# Autodesk Inventor assembly: Timing_Assy 4 Lanes
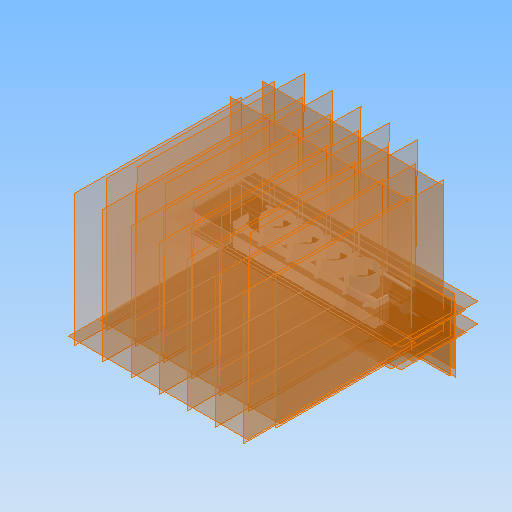
[picture p0: Inventor's stored thumbnail of the model, 512x512]
Saved by Autodesk Inventor 2018.1 (Build 221171000, 171)
## iProperties
Created: 2019-02-11
Part Number: Timing_Assy 4 Lanes
Document SubType Name: Assembly
Designer: James
Author: James
## Documents named in this file (9)
- C:\Users\admin\Desktop\Ball-Machine\Timing Gate\Timing - 4 Lanes\Timing_Assy 4 Lanes.iam
- C:\Users\admin\Desktop\Ball-Machine\Timing Gate\Nyloc Nut - M4.ipt
- C:\Users\admin\Desktop\Ball-Machine\Timing Gate\Socket Csk Screw - (A2) - M4 x  16.ipt
- C:\Users\admin\Desktop\Ball-Machine\Timing Gate\Timing_Angle Bracket.ipt
- C:\Users\admin\Desktop\Ball-Machine\Timing Gate\Socket Cap Screw - Standard - (A2) - M4 x 16.ipt
- C:\Users\admin\Desktop\Ball-Machine\Timing Gate\Timing_PVC Pipe.ipt
- C:\Users\admin\Desktop\Ball-Machine\Timing Gate\Timing - 4 Lanes\Timing_Backboard 4 Lanes.ipt
- C:\Users\admin\Desktop\Ball-Machine\Timing Gate\Timing - 4 Lanes\Timing_Assy_Lever Shaft 4 Lanes.iam
- C:\Users\admin\Desktop\Ball-Machine\Timing Gate\Timing - 4 Lanes\Timing_Assy_Star Shaft 4 Lanes.iam
## Components (33 placed, 8 different names)
1. Timing_Backboard 4 Lanes:1 — Flush:18, Mate:51, Mate:52, Tangent:1, Flush:19, Flush:20, Mate:55, Mate:56, Mate:59, Mate:60, Mate:67, Mate:68, Mate:69, Flush:27, Flush:28, Mate:74, Mate:75, Flush:29, Mate:82, Flush:30, Mate:83, Mate:84, Mate:85, Flush:31, Angle:2
2. Timing_Angle Bracket:1 — Mate:67, Mate:68, Mate:69, Flush:27, Flush:28, Mate:70, Mate:71, Mate:72, Mate:73, Flush:32, Flush:34
3. Nyloc Nut - M4:13 — Mate:74, Mate:76
4. Socket Cap Screw - Standard - (A2) - M4 x 16:3 — Mate:72, Mate:73, Mate:77
5. Nyloc Nut - M4:14 — Mate:75, Mate:77
6. Socket Cap Screw - Standard - (A2) - M4 x 16:4 — Mate:70, Mate:71, Mate:76
7. Timing_Angle Bracket:2 — Flush:29, Mate:82, Flush:30, Mate:83, Flush:33
8. Socket Cap Screw - Standard - (A2) - M4 x 16:5 — Mate:87
9. Socket Cap Screw - Standard - (A2) - M4 x 16:6 — Mate:86
10. Nyloc Nut - M4:15 — Mate:84, Mate:87
11. Nyloc Nut - M4:16 — Mate:85, Mate:86
12. Timing_Assy_Lever Shaft 4 Lanes:1 [sub-assembly] — Mate:88, Mate:89, Flush:31, Flush:32
13. Timing_Assy_Star Shaft 4 Lanes:1 [sub-assembly] — Flush:33, Flush:34, Mate:91, Angle:2, Mate:92
14. Timing_PVC Pipe:1 — Angle:1, Mate:51, Mate:52, Tangent:1, Mate:54
15. Nyloc Nut - M4:1 — Mate:58, Mate:59
16. Socket Csk Screw - (A2) - M4 x  16:1 — Mate:54, Mate:55, Flush:21, Mate:57
17. Socket Csk Screw - (A2) - M4 x  16:2 — Flush:21, Mate:56, Mate:58
18. Nyloc Nut - M4:2 — Mate:57, Mate:60
19. Timing_PVC Pipe:2
20. Nyloc Nut - M4:3
21. Socket Csk Screw - (A2) - M4 x  16:3
22. Socket Csk Screw - (A2) - M4 x  16:7
23. Nyloc Nut - M4:7
24. Timing_PVC Pipe:3
25. Nyloc Nut - M4:4
26. Socket Csk Screw - (A2) - M4 x  16:4
27. Socket Csk Screw - (A2) - M4 x  16:8
28. Nyloc Nut - M4:8
29. Timing_PVC Pipe:4
30. Nyloc Nut - M4:5
31. Socket Csk Screw - (A2) - M4 x  16:5
32. Socket Csk Screw - (A2) - M4 x  16:9
33. Nyloc Nut - M4:9
## Component patterns: (4 elements, first: Timing_PVC Pipe:1 + Nyloc Nut - M4:1 + Socket Csk Screw - (A2) - M4 x  16:1 + Socket Csk Screw - (A2) - M4 x  16:2 + Nyloc Nut - M4:2)
## Relationships (52: Mate 34, Flush 15, Angle 2, Tangent 1)
- Angle:1 (180 deg): Timing_PVC Pipe:1
- Flush:11 (-57.5 mm)
- Flush:12 (-5 mm)
- Flush:13 (30 mm)
- Flush:18: Timing_Backboard 4 Lanes:1
- Mate:51: Timing_Backboard 4 Lanes:1 ↔ Timing_PVC Pipe:1
- Mate:52: Timing_Backboard 4 Lanes:1 ↔ Timing_PVC Pipe:1
- Tangent:1: Timing_Backboard 4 Lanes:1 ↔ Timing_PVC Pipe:1
- Flush:19: Timing_Backboard 4 Lanes:1
- Flush:20: Timing_Backboard 4 Lanes:1
- Mate:54: Timing_PVC Pipe:1 ↔ Socket Csk Screw - (A2) - M4 x  16:1
- Mate:55 (-10.3 mm): Timing_Backboard 4 Lanes:1 ↔ Socket Csk Screw - (A2) - M4 x  16:1
- Flush:21: Socket Csk Screw - (A2) - M4 x  16:1 ↔ Socket Csk Screw - (A2) - M4 x  16:2
- Mate:56: Timing_Backboard 4 Lanes:1 ↔ Socket Csk Screw - (A2) - M4 x  16:2
- Mate:57: Socket Csk Screw - (A2) - M4 x  16:1 ↔ Nyloc Nut - M4:2
- Mate:58: Nyloc Nut - M4:1 ↔ Socket Csk Screw - (A2) - M4 x  16:2
- Mate:59: Timing_Backboard 4 Lanes:1 ↔ Nyloc Nut - M4:1
- Mate:60: Timing_Backboard 4 Lanes:1 ↔ Nyloc Nut - M4:2
- Mate:67: Timing_Backboard 4 Lanes:1 ↔ Timing_Angle Bracket:1
- Mate:68: Timing_Backboard 4 Lanes:1 ↔ Timing_Angle Bracket:1
- Mate:69: Timing_Backboard 4 Lanes:1 ↔ Timing_Angle Bracket:1
- Flush:27: Timing_Backboard 4 Lanes:1 ↔ Timing_Angle Bracket:1
- Flush:28: Timing_Backboard 4 Lanes:1 ↔ Timing_Angle Bracket:1
- Mate:70: Timing_Angle Bracket:1 ↔ Socket Cap Screw - Standard - (A2) - M4 x 16:4
- Mate:71: Timing_Angle Bracket:1 ↔ Socket Cap Screw - Standard - (A2) - M4 x 16:4
- Mate:72: Timing_Angle Bracket:1 ↔ Socket Cap Screw - Standard - (A2) - M4 x 16:3
- Mate:73: Timing_Angle Bracket:1 ↔ Socket Cap Screw - Standard - (A2) - M4 x 16:3
- Mate:74: Timing_Backboard 4 Lanes:1 ↔ Nyloc Nut - M4:13
- Mate:75: Timing_Backboard 4 Lanes:1 ↔ Nyloc Nut - M4:14
- Mate:76: Nyloc Nut - M4:13 ↔ Socket Cap Screw - Standard - (A2) - M4 x 16:4
- Mate:77: Socket Cap Screw - Standard - (A2) - M4 x 16:3 ↔ Nyloc Nut - M4:14
- [Mate]: Timing_Angle Bracket:2 ↔ Socket Cap Screw - Standard - (A2) - M4 x 16:6
- [Mate]: Timing_Angle Bracket:2 ↔ Socket Cap Screw - Standard - (A2) - M4 x 16:6
- [Mate]: Timing_Angle Bracket:2 ↔ Socket Cap Screw - Standard - (A2) - M4 x 16:5
- [Mate]: Timing_Angle Bracket:2 ↔ Socket Cap Screw - Standard - (A2) - M4 x 16:5
- Flush:29: Timing_Backboard 4 Lanes:1 ↔ Timing_Angle Bracket:2
- Mate:82: Timing_Backboard 4 Lanes:1 ↔ Timing_Angle Bracket:2
- Flush:30: Timing_Backboard 4 Lanes:1 ↔ Timing_Angle Bracket:2
- Mate:83: Timing_Backboard 4 Lanes:1 ↔ Timing_Angle Bracket:2
- Mate:84: Timing_Backboard 4 Lanes:1 ↔ Nyloc Nut - M4:15
- Mate:85: Timing_Backboard 4 Lanes:1 ↔ Nyloc Nut - M4:16
- Mate:86: Socket Cap Screw - Standard - (A2) - M4 x 16:6 ↔ Nyloc Nut - M4:16
- Mate:87: Socket Cap Screw - Standard - (A2) - M4 x 16:5 ↔ Nyloc Nut - M4:15
- Mate:88: Timing_Assy_Lever Shaft 4 Lanes:1
- Mate:89: Timing_Assy_Lever Shaft 4 Lanes:1
- Flush:31: Timing_Backboard 4 Lanes:1 ↔ Timing_Assy_Lever Shaft 4 Lanes:1
- Flush:32: Timing_Angle Bracket:1 ↔ Timing_Assy_Lever Shaft 4 Lanes:1
- Flush:33: Timing_Angle Bracket:2 ↔ Timing_Assy_Star Shaft 4 Lanes:1
- Flush:34: Timing_Angle Bracket:1 ↔ Timing_Assy_Star Shaft 4 Lanes:1
- Mate:91: Timing_Assy_Star Shaft 4 Lanes:1
- Angle:2 (0 deg): Timing_Backboard 4 Lanes:1 ↔ Timing_Assy_Star Shaft 4 Lanes:1
- Mate:92: Timing_Assy_Star Shaft 4 Lanes:1
## Named parameters: d139_d131 = 0 mm, d140_d132 = 0 mm, d141_d133 = 0 mm, d142_d134 = 0 mm
